# Autodesk Inventor assembly: intakeServoGear
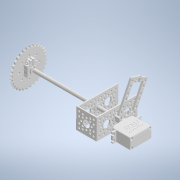
[picture p0: Inventor's stored thumbnail of the model, 180x180]
Saved by Autodesk Inventor 2020 (Build 240168000, 168)
## iProperties
Created: 2019-10-18
Part Number: intakeServoGear
Document SubType Name: Assembly
Designer: tdmp4
Author: tdmp4
## Documents named in this file (9)
- C:\Users\tdmp4\OneDrive\Documents\GitHub\CAD-2020\Intake\intakeServoGear.iam
- C:\Users\tdmp4\OneDrive\Documents\GitHub\CAD-2020\RevRobotics\REV-41-1097.ipt
- C:\Users\tdmp4\OneDrive\Documents\GitHub\CAD-2020\ServoCity\585484_1\585484.ipt
- C:\Users\tdmp4\OneDrive\Documents\GitHub\CAD-2020\ServoCity\535198.ipt
- C:\Users\tdmp4\OneDrive\Documents\GitHub\CAD-2020\ServoCity\634084.ipt
- C:\Users\tdmp4\OneDrive\Documents\GitHub\CAD-2020\ServoCity\525150_assembly (1)\525150 assembly.ipt
- C:\Users\tdmp4\OneDrive\Documents\GitHub\CAD-2020\ServoCity\615114.ipt
- C:\Users\tdmp4\OneDrive\Documents\GitHub\CAD-2020\ServoCity\545619 assembly.ipt
- C:\Users\tdmp4\OneDrive\Documents\GitHub\CAD-2020\ServoCity\575112\575112.ipt
## Components (9 placed, 8 different names)
1. REV-41-1097:1 — Mate:6, Mate:7, Mate:14
2. 585484:1 — Mate:1, Mate:2, Mate:3, Mate:4
3. 535198:1 — Mate:3, Mate:4, Mate:5, Mate:10
4. 535198:2 — Mate:1, Mate:2
5. 634084:1 — Mate:5, Mate:8, Mate:9, Insert:1
6. 525150 assembly:1 — Mate:6, Mate:7, Mate:8, Mate:9, Mate:10
7. 615114:1 — Mate:11, Mate:12, Mate:13
8. 545619 assembly:1 — Mate:11, Mate:12, Mate:13, Insert:1
9. 575112:1 — Mate:14
## Relationships (15: Mate 14, Insert 1)
- Mate:1: 585484:1 ↔ 535198:2
- Mate:2: 585484:1 ↔ 535198:2
- Mate:3: 585484:1 ↔ 535198:1
- Mate:4: 585484:1 ↔ 535198:1
- Mate:5: 535198:1 ↔ 634084:1
- Mate:6: REV-41-1097:1 ↔ 525150 assembly:1
- Mate:7: REV-41-1097:1 ↔ 525150 assembly:1
- Mate:8: 634084:1 ↔ 525150 assembly:1
- Mate:9: 634084:1 ↔ 525150 assembly:1
- Mate:10: 535198:1 ↔ 525150 assembly:1
- Mate:11: 615114:1 ↔ 545619 assembly:1
- Mate:12: 615114:1 ↔ 545619 assembly:1
- Mate:13: 615114:1 ↔ 545619 assembly:1
- Insert:1 (-12.7 mm): 634084:1 ↔ 545619 assembly:1
- Mate:14: REV-41-1097:1 ↔ 575112:1
